# Autodesk Inventor assembly: Canon_assem
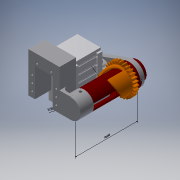
[picture p0: Inventor's stored thumbnail of the model, 180x180]
Saved by Autodesk Inventor 2018 (Build 220112000, 112)
## iProperties
Created: 2018-02-07
Part Number: Canon_assem
Material: Générique
Document SubType Name: Assembly
Designer: Mephiro
Author: Mephiro
## Documents named in this file (8)
- C:\Users\Mephiro\Google Drive\Robot_cup_3D\Canon_v3\Canon_assem.iam
- C:\Users\Mephiro\Google Drive\Robot_cup_3D\Canon_v3\canon.ipt
- C:\Users\Mephiro\Google Drive\Robot_cup_3D\Canon_v3\bottom.ipt
- C:\Users\Mephiro\Google Drive\Robot_cup_3D\Canon_v3\tige.ipt
- C:\Users\Mephiro\Google Drive\Robot_cup_3D\Canon_v3\charge_assem.iam
- C:\Users\Mephiro\Google Drive\Robot_cup_3D\Canon_v3\ax12.ipt
- C:\Users\Mephiro\Google Drive\Robot_cup_3D\Canon_v3\Engrenage_AX12.iam
- C:\Users\Mephiro\Google Drive\Robot_cup_3D\Canon_v3\support_axe.ipt
## Components (7 placed, 7 different names)
1. canon:1 — Logement:1, Placage:1, Placage:2, Placage:3, Placage:4
2. bottom:1 — Logement:1, Placage:1, Placage:5, Placage:6, Placage:7, Placage:10, Placage:11
3. tige:1 — Placage:2
4. charge_assem:1 [sub-assembly] — Placage:3, Placage:4, Tangente:1
5. ax12:1 — Placage:5, Placage:6, Placage:7, Placage:12, Placage:13
6. Engrenage_AX12:1 [sub-assembly] — Placage:12, Placage:13, Tangente:1, Placage:14, Placage:15
7. support_axe:1 — Placage:14, Placage:15
## Relationships (15: Mate 13, Insert 1, Tangent 1)
- Logement:1 [Insert]: canon:1 ↔ bottom:1
- Placage:1 [Mate]: canon:1 ↔ bottom:1
- Placage:2 [Mate]: canon:1 ↔ tige:1
- Placage:3 [Mate]: canon:1 ↔ charge_assem:1
- Placage:4 [Mate]: canon:1 ↔ charge_assem:1
- Placage:5 [Mate]: bottom:1 ↔ ax12:1
- Placage:6 [Mate]: bottom:1 ↔ ax12:1
- Placage:7 [Mate]: bottom:1 ↔ ax12:1
- Placage:10 [Mate]: bottom:1
- Placage:11 [Mate]: bottom:1
- Placage:12 [Mate]: ax12:1 ↔ Engrenage_AX12:1
- Placage:13 [Mate]: ax12:1 ↔ Engrenage_AX12:1
- Tangente:1: charge_assem:1 ↔ Engrenage_AX12:1
- Placage:14 [Mate]: Engrenage_AX12:1 ↔ support_axe:1
- Placage:15 [Mate]: Engrenage_AX12:1 ↔ support_axe:1
